# Autodesk Inventor assembly: MotorCoupling
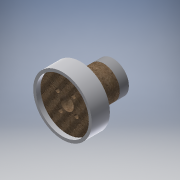
[picture p0: Inventor's stored thumbnail of the model, 180x180]
Saved by Autodesk Inventor 2016 (Build 200138000, 138)
## iProperties
Created: 2016-01-07
Part Number: MotorCoupling
Document SubType Name: Assembly
Designer: m2memari
Author: m2memari
## Documents named in this file (5)
- C:\MoDonGD\Jane\ShadowGame\ShadowGame\MotorCoupling.iam
- C:\MoDonGD\Jane\ShadowGame\ShadowGame\CouplingExtender.ipt
- C:\MoDonGD\Jane\ShadowGame\ShadowGame\CouplingHead.ipt
- C:\MoDonGD\Jane\ShadowGame\ShadowGame\CouplingScrew.ipt
- C:\MoDonGD\Jane\ShadowGame\ShadowGame\CouplingHead_Silicone.ipt
## Components (6 placed, 4 different names)
1. CouplingExtender:1 — Insert:1, Insert:2, Insert:3, Insert:4
2. CouplingHead:1 — Insert:7, Insert:8, Mate:1, Mate:2
3. CouplingScrew:1 — Insert:1, Insert:2
4. CouplingExtender:2 — Insert:5, Insert:6, Insert:7, Insert:8
5. CouplingExtender:3 — Insert:3, Insert:4, Insert:5, Insert:6
6. CouplingHead_Silicone:1 — Mate:1, Mate:2
## Relationships (10: Insert 8, Mate 2)
- Insert:1: CouplingExtender:1 ↔ CouplingScrew:1
- Insert:2: CouplingExtender:1 ↔ CouplingScrew:1
- Insert:3: CouplingExtender:1 ↔ CouplingExtender:3
- Insert:4: CouplingExtender:1 ↔ CouplingExtender:3
- Insert:5: CouplingExtender:2 ↔ CouplingExtender:3
- Insert:6: CouplingExtender:2 ↔ CouplingExtender:3
- Insert:7: CouplingHead:1 ↔ CouplingExtender:2
- Insert:8: CouplingHead:1 ↔ CouplingExtender:2
- Mate:1: CouplingHead:1 ↔ CouplingHead_Silicone:1
- Mate:2: CouplingHead:1 ↔ CouplingHead_Silicone:1
